# Autodesk Inventor assembly: coil winder V2
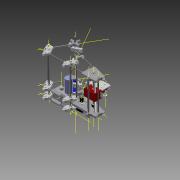
[picture p0: Inventor's stored thumbnail of the model, 180x180]
Saved by Autodesk Inventor 2013 (Build 170138000, 138)
## iProperties
Created: 2013-01-01
Part Number: coil winder V2
Document SubType Name: Assembly
Designer: Nico
Mass: 1980.92 g
Surface Area: 5858.81 cm^2
Volume: 1384.16 cm^3
Density: 1.43114 g/cm^3
Author: Nico
## Documents named in this file (37)
- D:\Documents\Inventor\Coil winder\IAM files\coil winder V2.iam
- D:\Documents\Inventor\Coil winder\IAM files\Winder Assembly 1.iam
- D:\Documents\Inventor\Coil winder\Drive thread.ipt
- D:\Documents\Inventor\Coil winder\IPT files\Washer M8.ipt
- D:\Documents\Inventor\Coil winder\IPT files\Half Nut M8.ipt
- D:\Documents\Inventor\Coil winder\IPT files\Pulley HTD 3-40-7.8.ipt
- D:\Documents\Inventor\Coil winder\IPT files\DC Motor stand V2.ipt
- D:\Documents\Inventor\Coil winder\IAM files\Nut+Washer M8.iam
- D:\Documents\Inventor\Coil winder\IAM files\Motor assembly V2.iam
- D:\Documents\Inventor\Coil winder\IPT files\carre Washer M8.ipt
- D:\Documents\Inventor\Coil winder\IPT files\bolt M4 x 10 nickel plated.ipt
- D:\Documents\Inventor\Coil winder\IPT files\connect stepper.ipt
- D:\Documents\Inventor\Coil winder\coil winder V2\Design Accelerator\Compress Spring1.iam
- D:\Documents\Inventor\Coil winder\IPT files\Sensor stand.ipt
- D:\Documents\Inventor\Coil winder\IPT files\optical sensor pcb.ipt
- D:\Documents\Inventor\Coil winder\IPT files\Vertex Bottom tensioner left.ipt
- D:\Documents\Inventor\Coil winder\IPT files\slide rod.ipt
- D:\Documents\Inventor\Coil winder\IAM files\Wire tension assembly.iam
- D:\Documents\Inventor\Coil winder\IPT files\608ZZ bearing.ipt
- D:\Documents\Inventor\Coil winder\IPT files\Nema 17 stepper motor.ipt
- D:\Documents\Inventor\Coil winder\Drive thread\Thread rod M8 x 100 mm.ipt
- D:\Documents\Inventor\Coil winder\Drive thread\Thread rod M8 x 300 mm.ipt
- D:\Documents\Inventor\Coil winder\Drive thread\Thread rod M8 x 190 mm.ipt
- D:\Documents\Inventor\Coil winder\Drive thread\Thread rod M8 x 250 mm.ipt
- D:\Documents\Inventor\Coil winder\IPT files\Vertex Bottom tensioner right.ipt
- D:\Documents\Inventor\Coil winder\Drive thread\Thread rod M8 x 380 mm.ipt
- D:\Documents\Inventor\Coil winder\Drive thread\Thread rod M8 x 230 mm.ipt
- D:\Documents\Inventor\Coil winder\IPT files\Stepper Pulley HTD 3 x 6 x 20.ipt
- D:\Documents\Inventor\Coil winder\IPT files\bolt M3 x 12 nickel plated.ipt
- D:\Documents\Inventor\Coil winder\IPT files\Washer M3 nickel plated.ipt
- D:\Documents\Inventor\Coil winder\IPT files\Tensioner Pulley HTD 3 x 6 x 20.ipt
- D:\Documents\Inventor\Coil winder\IPT files\Coil Coupling_1.ipt
- D:\Documents\Inventor\Coil winder\IPT files\Coil Coupling_2.ipt
- D:\Documents\Inventor\Coil winder\Drive thread\8mm thread 150 mm long.ipt
- D:\Documents\Inventor\Coil winder\IPT files\Drive thread.ipt
- D:\Documents\Inventor\Coil winder\IPT files\coil tightner.ipt
- Stepper Pulley HTD 3 x 6 x 20.ipt
## Components (151 placed, 32 different names)
1. Winder Assembly 1:1 [sub-assembly] — Mate:1, Mate:2, Mate:17, Mate:18, Mate:46, Mate:47, Mate:60, Mate:61, Mate:65, Mate:88, Mate:89, Mate:96, Mate:98, Mate:145, Flush:8, Mate:151, Mate:152, Mate:179, Mate:181, Mate:212, Mate:216, Mate:227, Mate:228
2. Winder Assembly 1:2 [sub-assembly] — Mate:1, Mate:2, Mate:4, Mate:19, Mate:20, Mate:30, Mate:42, Mate:43, Mate:62, Mate:63, Mate:64, Mate:72, Mate:73, Mate:80, Mate:81, Mate:180, Mate:210, Mate:215, Mate:225, Mate:226
3. Thread rod M8 x 100 mm:1 — Mate:4, Mate:13, Mate:14, Mate:15, Mate:16, Flush:1, Mate:21, Mate:27, Mate:100, Mate:114, Mate:137
4. Washer M8:1 — Mate:5, Mate:9, Mate:17
5. Washer M8:2 — Mate:6, Mate:12, Mate:20
6. Washer M8:3 — Mate:7, Mate:10, Mate:19
7. Washer M8:4 — Mate:8, Mate:11, Mate:18
8. Half Nut M8:1 — Mate:5, Mate:9, Mate:13
9. Half Nut M8:2 — Mate:6, Mate:12, Mate:14, Flush:1
10. Half Nut M8:3 — Mate:7, Mate:10, Mate:15, Mate:29
11. Half Nut M8:4 — Mate:8, Mate:11, Mate:16, Mate:140
12. Pulley HTD 3-40-7.8:1 — Mate:21, Mate:28, Mate:115
13. Washer M8:5 — Mate:23, Mate:25, Mate:115
14. Washer M8:6 — Mate:28, Mate:29, Mate:114
15. Half Nut M8:5 — Mate:23, Mate:25, Mate:27
16. Thread rod M8 x 300 mm:3 — Mate:30, Mate:52, Mate:53, Mate:58, Mate:59, Flush:3, Mate:99, Mate:126, Mate:127
17. Washer M8:7 — Mate:33, Mate:38, Mate:43
18. Washer M8:8 — Mate:35, Mate:37, Mate:47
19. Washer M8:9 — Mate:48, Mate:49, Mate:60
20. Washer M8:10 — Mate:54, Mate:55, Mate:61
21. Washer M8:11 — Mate:32, Mate:39, Mate:42
22. Washer M8:12 — Mate:34, Mate:36, Mate:46
23. Washer M8:13 — Mate:50, Mate:51, Mate:63
24. Washer M8:14 — Mate:56, Mate:57, Mate:62
25. Half Nut M8:6 — Mate:32, Mate:39
26. Half Nut M8:7 — Mate:33, Mate:38
27. Half Nut M8:8 — Mate:34, Mate:36
28. Half Nut M8:9 — Mate:35, Mate:37
29. Half Nut M8:10 — Mate:50, Mate:51, Mate:52, Flush:3
30. Half Nut M8:11 — Mate:48, Mate:49, Mate:53
31. Half Nut M8:12 — Mate:54, Mate:55, Mate:59
32. Half Nut M8:13 — Mate:56, Mate:57, Mate:58
33. Thread rod M8 x 190 mm:4 — Mate:64, Mate:70, Mate:71, Flush:4, Mate:78, Mate:79, Mate:102
34. Thread rod M8 x 380 mm:5 — Mate:65, Mate:86, Mate:87, Mate:95, Mate:97, Mate:101, Mate:282, Flush:33, Mate:429, Flush:34
35. Half Nut M8:14 — Mate:75, Mate:76, Mate:78
36. Half Nut M8:15 — Mate:74, Mate:77, Mate:79
37. Half Nut M8:16 — Mate:66, Mate:69, Mate:70
38. Half Nut M8:17 — Mate:67, Mate:68, Mate:71, Flush:4
39. Washer M8:15 — Mate:75, Mate:76, Mate:80
40. Washer M8:16 — Mate:74, Mate:77, Mate:81
41. Washer M8:17 — Mate:66, Mate:69, Mate:72
42. Washer M8:18 — Mate:67, Mate:68, Mate:73
43. Washer M8:19 — Mate:91, Mate:92, Mate:98
44. Washer M8:20 — Mate:90, Mate:93, Mate:96
45. Washer M8:21 — Mate:82, Mate:84, Mate:88
46. Washer M8:22 — Mate:83, Mate:85, Mate:89
47. Half Nut M8:18 — Mate:91, Mate:92, Mate:97, Flush:33
48. Half Nut M8:19 — Mate:90, Mate:93, Mate:95
49. Half Nut M8:20 — Mate:82, Mate:84, Mate:87
50. Half Nut M8:21 — Mate:83, Mate:85, Mate:86
51. Winder Assembly 1:3 [sub-assembly] — Mate:99, Mate:100, Mate:117, Mate:122, Mate:123, Mate:124, Mate:125, Mate:130, Mate:131, Mate:132, Mate:133, Mate:165, Mate:169, Mate:182, Mate:184, Mate:206, Mate:208, Mate:219, Mate:220, Mate:392, Mate:394, Mate:396
52. DC Motor stand V2:1 — Mate:101, Mate:102, Mate:103, Mate:105, Mate:106, Mate:107, Mate:108, Mate:109, Mate:110, Mate:113, Mate:422, Mate:423
53. Nut+Washer M8:1 [sub-assembly] — Mate:105, Mate:107
54. Nut+Washer M8:2 [sub-assembly] — Mate:106, Mate:109
55. Nut+Washer M8:3 [sub-assembly] — Mate:104, Mate:110
56. Nut+Washer M8:4 [sub-assembly] — Mate:103, Mate:104, Mate:108
57. Motor assembly V2:1 [sub-assembly] — Mate:113, Mate:422, Mate:423, Mate:424, Mate:425, Mate:426, Mate:427
58. Thread rod M8 x 380 mm:6 — Mate:117, Mate:118, Mate:119, Mate:120, Mate:121, Flush:6, Mate:231, Mate:232, Mate:402
59. Nut+Washer M8:5 [sub-assembly] — Mate:118, Mate:125
60. Nut+Washer M8:6 [sub-assembly] — Mate:120, Mate:123, Flush:6
61. Nut+Washer M8:7 [sub-assembly] — Mate:121, Mate:122
62. Nut+Washer M8:8 [sub-assembly] — Mate:119, Mate:124
63. Nut+Washer M8:9 [sub-assembly] — Mate:126, Mate:133
64. Nut+Washer M8:10 [sub-assembly] — Mate:127, Mate:132
65. Nut+Washer M8:11 [sub-assembly] — Mate:131, Mate:183, Flush:19
66. Nut+Washer M8:12 [sub-assembly] — Mate:130, Mate:287
67. Coil Coupling_1:1 — Mate:470
68. Half Nut M8:22 — Mate:137, Mate:138
69. Washer M8:23 — Mate:138, Mate:140
70. Bolt M4 x 10 nickel plated:1 — Mate:424, Mate:426
71. Bolt M4 x 10 nickel plated:2 — Mate:425, Mate:427
72. connect stepper:1 — Mate:145, Flush:8, Mate:146, Mate:148, Mate:149, Mate:150, Mate:153, Mate:154, Flush:32
73. Thread rod M8 x 230 mm:7 — Mate:146, Mate:147, Flush:9, Mate:274, Mate:281
74. Nut+Washer M8:13 [sub-assembly] — Mate:147, Mate:150
75. Nut+Washer M8:14 [sub-assembly] — Mate:148, Mate:149, Flush:9
76. Nut+Washer M8:15 [sub-assembly] — Mate:152, Mate:153
77. Nut+Washer M8:16 [sub-assembly] — Mate:151, Mate:154
78. connect stepper:2 — Mate:392, Mate:395, Mate:397, Mate:398, Mate:399, Mate:400, Flush:32
79. Thread rod M8 x 230 mm:8 — Mate:157, Mate:158, Flush:12, Mate:233, Mate:398, Mate:401, Mate:404
80. Nut+Washer M8:17 [sub-assembly] — Mate:157, Mate:400
81. Nut+Washer M8:18 [sub-assembly] — Mate:158, Flush:12, Mate:399
82. Nut+Washer M8:19 [sub-assembly] — Mate:394, Mate:397
83. Nut+Washer M8:20 [sub-assembly] — Mate:395, Mate:396
84. 8mm thread 150 mm long:16 — Mate:165, Mate:166, Mate:172, Mate:173, Mate:175, Mate:468, Mate:469, Mate:471
85. Nut+Washer M8:21 [sub-assembly] — Mate:166, Mate:169
86. Coil Coupling_1:2
87. Half Nut M8:23 — Mate:172
88. Washer M8:24 — Mate:173, Flush:14
89. Compress Spring:1 [sub-assembly] — Mate:175, Flush:14
90. Sensor stand:1 — Mate:179, Mate:180
91. optical sensor pcb:1
92. Thread rod M8 x 300 mm:10 — Mate:181, Mate:205, Flush:16, Mate:207, Mate:209, Mate:211, Mate:213, Mate:214, Flush:17
93. Thread rod M8 x 300 mm:11 — Mate:182, Mate:217, Mate:218, Flush:18, Mate:221, Mate:222, Mate:223, Mate:224, Flush:20
94. Thread rod M8 x 300 mm:12 — Mate:183, Mate:184, Flush:19, Mate:287
95. Vertex Bottom tensioner left:1 — Mate:401, Mate:402, Mate:403, Mate:405, Mate:406, Mate:407, Mate:408, Mate:409, Mate:410, Mate:411, Mate:412, Mate:413, Mate:414, Mate:415, Mate:416, Mate:417, Mate:420, Mate:421
96. Thread rod M8 x 250 mm:13 — Mate:238, Mate:241, Mate:244, Flush:23, Mate:264, Mate:269, Mate:412
97. slide rod:1 — Mate:410, Mate:415, Mate:419
98. slide rod:2 — Mate:411, Mate:416, Mate:418
99. 608ZZ bearing:1 — Mate:204, Mate:249, Mate:250, Mate:414
100. 608ZZ bearing:2 — Mate:279, Mate:280, Mate:430, Mate:431
101. Thread rod M8 x 250 mm:14 — Mate:204, Mate:247, Mate:248, Flush:24, Mate:272, Mate:275, Mate:409, Mate:430, Mate:434, Mate:444, Mate:445
102. Nut+Washer M8:23 [sub-assembly] — Mate:205, Mate:206, Flush:16
103. Nut+Washer M8:24 [sub-assembly] — Mate:218, Mate:220
104. Nut+Washer M8:25 [sub-assembly] — Mate:207, Mate:208
105. Nut+Washer M8:26 [sub-assembly] — Mate:217, Mate:219, Flush:18
106. Nut+Washer M8:27 [sub-assembly] — Mate:209, Mate:210, Flush:17
107. Nut+Washer M8:28 [sub-assembly] — Mate:211, Mate:212
108. Nut+Washer M8:29 [sub-assembly] — Mate:214, Mate:215
109. Nut+Washer M8:30 [sub-assembly] — Mate:213, Mate:216
110. Nut+Washer M8:31 [sub-assembly] — Mate:221, Mate:227
111. Nut+Washer M8:32 [sub-assembly] — Mate:222, Mate:228
112. Nut+Washer M8:33 [sub-assembly] — Mate:223, Mate:226, Flush:20
113. Nut+Washer M8:34 [sub-assembly] — Mate:224, Mate:225
114. Nut+Washer M8:35 [sub-assembly] — Mate:404, Mate:405
115. Nut+Washer M8:36 [sub-assembly] — Mate:231, Mate:421
116. Nut+Washer M8:37 [sub-assembly] — Mate:232, Mate:403
117. Nut+Washer M8:38 [sub-assembly] — Mate:233, Mate:406
118. Thread rod M8 x 250 mm:15 — Mate:239, Mate:242, Flush:22, Mate:266, Mate:268, Mate:407
119. Nut+Washer M8:39 [sub-assembly] — Mate:238, Flush:23, Mate:413
120. Nut+Washer M8:40 [sub-assembly] — Mate:239, Flush:22, Mate:417
121. Nut+Washer M8:41 [sub-assembly] — Mate:241, Mate:244, Mate:420
122. Nut+Washer M8:42 [sub-assembly] — Mate:242, Mate:408
123. Nut+Washer M8:43 [sub-assembly] — Mate:247, Mate:250, Flush:24
124. Nut+Washer M8:44 [sub-assembly] — Mate:248, Mate:249
125. Nut+Washer M8:45 [sub-assembly] — Mate:266, Mate:435
126. Nut+Washer M8:46 [sub-assembly] — Mate:264, Mate:438, Mate:439
127. Nut+Washer M8:47 [sub-assembly] — Mate:269, Mate:437
128. Nut+Washer M8:48 [sub-assembly] — Mate:268, Mate:436
129. Nut+Washer M8:49 [sub-assembly] — Mate:274
130. Nut+Washer M8:51 [sub-assembly] — Mate:275, Mate:280
131. Nut+Washer M8:52 [sub-assembly] — Mate:272, Mate:279
132. Nut+Washer M8:53 [sub-assembly] — Mate:281, Mate:433
133. Nut+Washer M8:54 [sub-assembly] — Mate:282, Mate:432, Flush:34
134. Wire tension assembly:1 [sub-assembly] — Mate:418, Mate:419
135. Nema 17 stepper motor:1 — Mate:434, Flush:35, Mate:449, Mate:462, Mate:463, Mate:464, Mate:465
136. Vertex Bottom tensioner right:1 — Mate:429, Mate:431, Mate:432, Mate:433, Mate:435, Mate:436, Mate:437, Mate:438, Mate:439, Flush:35, Mate:458, Mate:459, Mate:460, Mate:461
137. Stepper Pulley HTD 3 x 6 x 20:1 — Mate:449
138. Tensioner Pulley HTD 3 x 6 x 20:1
139. Nut+Washer M8:55 [sub-assembly] — Mate:445
140. Nut+Washer M8:56 [sub-assembly] — Mate:444
141. bolt M3 x 12 nickel plated:1 — Mate:453, Mate:456, Mate:463
142. bolt M3 x 12 nickel plated:2 — Mate:450, Mate:455, Mate:462
143. bolt M3 x 12 nickel plated:3 — Mate:451, Mate:454, Mate:465
144. bolt M3 x 12 nickel plated:4 — Mate:452, Mate:457, Mate:464
145. Washer M3 Nickel plated:1 — Mate:453, Mate:456, Mate:459
146. Washer M3 Nickel plated:2 — Mate:452, Mate:457, Mate:460
147. Washer M3 Nickel plated:3 — Mate:451, Mate:454, Mate:461
148. Washer M3 Nickel plated:4 — Mate:450, Mate:455, Mate:458
149. Coil Coupling_2:1 — Mate:468
150. Coil Coupling_2:2 — Mate:469, Mate:470
151. coil tightner:1 — Mate:471
## Relationships (286: Mate 266, Flush 20)
- Mate:1: Winder Assembly 1:1 ↔ Winder Assembly 1:2
- Mate:2: Winder Assembly 1:1 ↔ Winder Assembly 1:2
- Mate:4: Winder Assembly 1:2 ↔ Thread rod M8 x 100 mm:1
- Mate:5: Washer M8:1 ↔ Half Nut M8:1
- Mate:6: Washer M8:2 ↔ Half Nut M8:2
- Mate:7: Washer M8:3 ↔ Half Nut M8:3
- Mate:8: Washer M8:4 ↔ Half Nut M8:4
- Mate:9: Washer M8:1 ↔ Half Nut M8:1
- Mate:10: Washer M8:3 ↔ Half Nut M8:3
- Mate:11: Washer M8:4 ↔ Half Nut M8:4
- Mate:12: Washer M8:2 ↔ Half Nut M8:2
- Mate:13: Thread rod M8 x 100 mm:1 ↔ Half Nut M8:1
- Mate:14: Thread rod M8 x 100 mm:1 ↔ Half Nut M8:2
- Mate:15: Thread rod M8 x 100 mm:1 ↔ Half Nut M8:3
- Mate:16: Thread rod M8 x 100 mm:1 ↔ Half Nut M8:4
- Mate:17: Winder Assembly 1:1 ↔ Washer M8:1
- Mate:18: Winder Assembly 1:1 ↔ Washer M8:4
- Mate:19: Winder Assembly 1:2 ↔ Washer M8:3
- Mate:20: Winder Assembly 1:2 ↔ Washer M8:2
- Flush:1 (-2 mm): Thread rod M8 x 100 mm:1 ↔ Half Nut M8:2
- Mate:21: Thread rod M8 x 100 mm:1 ↔ Pulley HTD 3-40-7.8:1
- Mate:23: Washer M8:5 ↔ Half Nut M8:5
- Mate:25: Washer M8:5 ↔ Half Nut M8:5
- Mate:27: Thread rod M8 x 100 mm:1 ↔ Half Nut M8:5
- Mate:28: Pulley HTD 3-40-7.8:1 ↔ Washer M8:6
- Mate:29: Half Nut M8:3 ↔ Washer M8:6
- Mate:30: Winder Assembly 1:2 ↔ Thread rod M8 x 300 mm:3
- Mate:32: Washer M8:11 ↔ Half Nut M8:6
- Mate:33: Washer M8:7 ↔ Half Nut M8:7
- Mate:34: Washer M8:12 ↔ Half Nut M8:8
- Mate:35: Washer M8:8 ↔ Half Nut M8:9
- Mate:36: Washer M8:12 ↔ Half Nut M8:8
- Mate:37: Washer M8:8 ↔ Half Nut M8:9
- Mate:38: Washer M8:7 ↔ Half Nut M8:7
- Mate:39: Washer M8:11 ↔ Half Nut M8:6
- Mate:42: Winder Assembly 1:2 ↔ Washer M8:11
- Mate:43: Winder Assembly 1:2 ↔ Washer M8:7
- Mate:46: Winder Assembly 1:1 ↔ Washer M8:12
- Mate:47: Winder Assembly 1:1 ↔ Washer M8:8
- Mate:48: Washer M8:9 ↔ Half Nut M8:11
- Mate:49: Washer M8:9 ↔ Half Nut M8:11
- Mate:50: Washer M8:13 ↔ Half Nut M8:10
- Mate:51: Washer M8:13 ↔ Half Nut M8:10
- Mate:52: Thread rod M8 x 300 mm:3 ↔ Half Nut M8:10
- Mate:53: Thread rod M8 x 300 mm:3 ↔ Half Nut M8:11
- Mate:54: Washer M8:10 ↔ Half Nut M8:12
- Mate:55: Washer M8:10 ↔ Half Nut M8:12
- Mate:56: Washer M8:14 ↔ Half Nut M8:13
- Mate:57: Washer M8:14 ↔ Half Nut M8:13
- Mate:58: Thread rod M8 x 300 mm:3 ↔ Half Nut M8:13
- Mate:59: Thread rod M8 x 300 mm:3 ↔ Half Nut M8:12
- Mate:60: Winder Assembly 1:1 ↔ Washer M8:9
- Mate:61: Winder Assembly 1:1 ↔ Washer M8:10
- Mate:62: Winder Assembly 1:2 ↔ Washer M8:14
- Mate:63: Winder Assembly 1:2 ↔ Washer M8:13
- Flush:3 (-2 mm): Thread rod M8 x 300 mm:3 ↔ Half Nut M8:10
- Mate:64: Winder Assembly 1:2 ↔ Thread rod M8 x 190 mm:4
- Mate:65: Winder Assembly 1:1 ↔ Thread rod M8 x 380 mm:5
- Mate:66: Half Nut M8:16 ↔ Washer M8:17
- Mate:67: Half Nut M8:17 ↔ Washer M8:18
- Mate:68: Half Nut M8:17 ↔ Washer M8:18
- Mate:69: Half Nut M8:16 ↔ Washer M8:17
- Mate:70: Thread rod M8 x 190 mm:4 ↔ Half Nut M8:16
- Mate:71: Thread rod M8 x 190 mm:4 ↔ Half Nut M8:17
- Mate:72: Winder Assembly 1:2 ↔ Washer M8:17
- Mate:73: Winder Assembly 1:2 ↔ Washer M8:18
- Flush:4 (-2 mm): Thread rod M8 x 190 mm:4 ↔ Half Nut M8:17
- Mate:74: Half Nut M8:15 ↔ Washer M8:16
- Mate:75: Half Nut M8:14 ↔ Washer M8:15
- Mate:76: Half Nut M8:14 ↔ Washer M8:15
- Mate:77: Half Nut M8:15 ↔ Washer M8:16
- Mate:78: Thread rod M8 x 190 mm:4 ↔ Half Nut M8:14
- Mate:79: Thread rod M8 x 190 mm:4 ↔ Half Nut M8:15
- Mate:80: Winder Assembly 1:2 ↔ Washer M8:15
- Mate:81: Winder Assembly 1:2 ↔ Washer M8:16
- Mate:82: Washer M8:21 ↔ Half Nut M8:20
- Mate:83: Washer M8:22 ↔ Half Nut M8:21
- Mate:84: Washer M8:21 ↔ Half Nut M8:20
- Mate:85: Washer M8:22 ↔ Half Nut M8:21
- Mate:86: Thread rod M8 x 380 mm:5 ↔ Half Nut M8:21
- Mate:87: Thread rod M8 x 380 mm:5 ↔ Half Nut M8:20
- Mate:88: Winder Assembly 1:1 ↔ Washer M8:21
- Mate:89: Winder Assembly 1:1 ↔ Washer M8:22
- Mate:90: Washer M8:20 ↔ Half Nut M8:19
- Mate:91: Washer M8:19 ↔ Half Nut M8:18
- Mate:92: Washer M8:19 ↔ Half Nut M8:18
- Mate:93: Washer M8:20 ↔ Half Nut M8:19
- Mate:95: Thread rod M8 x 380 mm:5 ↔ Half Nut M8:19
- Mate:96: Winder Assembly 1:1 ↔ Washer M8:20
- Mate:97: Thread rod M8 x 380 mm:5 ↔ Half Nut M8:18
- Mate:98: Winder Assembly 1:1 ↔ Washer M8:19
- Mate:99: Thread rod M8 x 300 mm:3 ↔ Winder Assembly 1:3
- Mate:100: Thread rod M8 x 100 mm:1 ↔ Winder Assembly 1:3
- Mate:101: Thread rod M8 x 380 mm:5 ↔ DC Motor stand V2:1
- Mate:102: Thread rod M8 x 190 mm:4 ↔ DC Motor stand V2:1
- Mate:103: DC Motor stand V2:1 ↔ Nut+Washer M8:4
- Mate:104: Nut+Washer M8:3 ↔ Nut+Washer M8:4
- Mate:105: DC Motor stand V2:1 ↔ Nut+Washer M8:1
- Mate:106: DC Motor stand V2:1 ↔ Nut+Washer M8:2
- Mate:107: DC Motor stand V2:1 ↔ Nut+Washer M8:1
- Mate:108: DC Motor stand V2:1 ↔ Nut+Washer M8:4
- Mate:109: DC Motor stand V2:1 ↔ Nut+Washer M8:2
- Mate:110: DC Motor stand V2:1 ↔ Nut+Washer M8:3
- Mate:113: DC Motor stand V2:1 ↔ Motor assembly V2:1
- Mate:114: Thread rod M8 x 100 mm:1 ↔ Washer M8:6
- Mate:115: Pulley HTD 3-40-7.8:1 ↔ Washer M8:5
- Mate:117: Winder Assembly 1:3 ↔ Thread rod M8 x 380 mm:6
- Mate:118: Thread rod M8 x 380 mm:6 ↔ Nut+Washer M8:5
- Mate:119: Thread rod M8 x 380 mm:6 ↔ Nut+Washer M8:8
- Mate:120: Thread rod M8 x 380 mm:6 ↔ Nut+Washer M8:6
- Mate:121: Thread rod M8 x 380 mm:6 ↔ Nut+Washer M8:7
- Mate:122: Winder Assembly 1:3 ↔ Nut+Washer M8:7
- Mate:123: Winder Assembly 1:3 ↔ Nut+Washer M8:6
- Mate:124: Winder Assembly 1:3 ↔ Nut+Washer M8:8
- Mate:125: Winder Assembly 1:3 ↔ Nut+Washer M8:5
- Flush:6 (-2 mm): Thread rod M8 x 380 mm:6 ↔ Nut+Washer M8:6
- Mate:126: Thread rod M8 x 300 mm:3 ↔ Nut+Washer M8:9
- Mate:127: Thread rod M8 x 300 mm:3 ↔ Nut+Washer M8:10
- Mate:130: Winder Assembly 1:3 ↔ Nut+Washer M8:12
- Mate:131: Winder Assembly 1:3 ↔ Nut+Washer M8:11
- Mate:132: Winder Assembly 1:3 ↔ Nut+Washer M8:10
- Mate:133: Winder Assembly 1:3 ↔ Nut+Washer M8:9
- Mate:137: Thread rod M8 x 100 mm:1 ↔ Half Nut M8:22
- Mate:138: Half Nut M8:22 ↔ Washer M8:23
- Mate:140: Half Nut M8:4 ↔ Washer M8:23
- Mate:145: Winder Assembly 1:1 ↔ connect stepper:1
- Flush:8 (-0.5 mm): Winder Assembly 1:1 ↔ connect stepper:1
- Mate:146: connect stepper:1 ↔ Thread rod M8 x 230 mm:7
- Mate:147: Thread rod M8 x 230 mm:7 ↔ Nut+Washer M8:13
- Mate:148: connect stepper:1 ↔ Nut+Washer M8:14
- Mate:149: connect stepper:1 ↔ Nut+Washer M8:14
- Mate:150: connect stepper:1 ↔ Nut+Washer M8:13
- Flush:9 (-2 mm): Thread rod M8 x 230 mm:7 ↔ Nut+Washer M8:14
- Mate:151: Winder Assembly 1:1 ↔ Nut+Washer M8:16
- Mate:152: Winder Assembly 1:1 ↔ Nut+Washer M8:15
- Mate:153: connect stepper:1 ↔ Nut+Washer M8:15
- Mate:154: connect stepper:1 ↔ Nut+Washer M8:16
- Mate:157: Thread rod M8 x 230 mm:8 ↔ Nut+Washer M8:17
- Mate:158: Thread rod M8 x 230 mm:8 ↔ Nut+Washer M8:18
- Flush:12 (-2 mm): Thread rod M8 x 230 mm:8 ↔ Nut+Washer M8:18
- Mate:165: Winder Assembly 1:3 ↔ 8mm thread 150 mm long:16
- Mate:166: 8mm thread 150 mm long:16 ↔ Nut+Washer M8:21
- Mate:169: Winder Assembly 1:3 ↔ Nut+Washer M8:21
- Mate:172: 8mm thread 150 mm long:16 ↔ Half Nut M8:23
- Mate:173: 8mm thread 150 mm long:16 ↔ Washer M8:24
- Mate:175: 8mm thread 150 mm long:16 ↔ Compress Spring:1
- Flush:14: Washer M8:24 ↔ Compress Spring:1
- Mate:179: Winder Assembly 1:1 ↔ Sensor stand:1
- Mate:180: Winder Assembly 1:2 ↔ Sensor stand:1
- Mate:181: Winder Assembly 1:1 ↔ Thread rod M8 x 300 mm:10
- Mate:182: Winder Assembly 1:3 ↔ Thread rod M8 x 300 mm:11
- Mate:183: Nut+Washer M8:11 ↔ Thread rod M8 x 300 mm:12
- Mate:184: Winder Assembly 1:3 ↔ Thread rod M8 x 300 mm:12
- Mate:204: 608ZZ bearing:1 ↔ Thread rod M8 x 250 mm:14
- Mate:205: Thread rod M8 x 300 mm:10 ↔ Nut+Washer M8:23
- Mate:206: Winder Assembly 1:3 ↔ Nut+Washer M8:23
- Flush:16 (-2 mm): Thread rod M8 x 300 mm:10 ↔ Nut+Washer M8:23
- Mate:207: Thread rod M8 x 300 mm:10 ↔ Nut+Washer M8:25
- Mate:208: Winder Assembly 1:3 ↔ Nut+Washer M8:25
- Mate:209: Thread rod M8 x 300 mm:10 ↔ Nut+Washer M8:27
- Mate:210: Winder Assembly 1:2 ↔ Nut+Washer M8:27
- Mate:211: Thread rod M8 x 300 mm:10 ↔ Nut+Washer M8:28
- Mate:212: Winder Assembly 1:1 ↔ Nut+Washer M8:28
- Mate:213: Thread rod M8 x 300 mm:10 ↔ Nut+Washer M8:30
- Mate:214: Thread rod M8 x 300 mm:10 ↔ Nut+Washer M8:29
- Mate:215: Winder Assembly 1:2 ↔ Nut+Washer M8:29
- Mate:216: Winder Assembly 1:1 ↔ Nut+Washer M8:30
- Flush:17 (-2 mm): Thread rod M8 x 300 mm:10 ↔ Nut+Washer M8:27
- Mate:217: Thread rod M8 x 300 mm:11 ↔ Nut+Washer M8:26
- Mate:218: Thread rod M8 x 300 mm:11 ↔ Nut+Washer M8:24
- Mate:219: Winder Assembly 1:3 ↔ Nut+Washer M8:26
- Mate:220: Winder Assembly 1:3 ↔ Nut+Washer M8:24
- Flush:18 (-2 mm): Thread rod M8 x 300 mm:11 ↔ Nut+Washer M8:26
- Flush:19 (-2 mm): Nut+Washer M8:11 ↔ Thread rod M8 x 300 mm:12
- Mate:221: Thread rod M8 x 300 mm:11 ↔ Nut+Washer M8:31
- Mate:222: Thread rod M8 x 300 mm:11 ↔ Nut+Washer M8:32
- Mate:223: Thread rod M8 x 300 mm:11 ↔ Nut+Washer M8:33
- Mate:224: Thread rod M8 x 300 mm:11 ↔ Nut+Washer M8:34
- Mate:225: Winder Assembly 1:2 ↔ Nut+Washer M8:34
- Mate:226: Winder Assembly 1:2 ↔ Nut+Washer M8:33
- Flush:20 (-2 mm): Thread rod M8 x 300 mm:11 ↔ Nut+Washer M8:33
- Mate:227: Winder Assembly 1:1 ↔ Nut+Washer M8:31
- Mate:228: Winder Assembly 1:1 ↔ Nut+Washer M8:32
- Mate:231: Thread rod M8 x 380 mm:6 ↔ Nut+Washer M8:36
- Mate:232: Thread rod M8 x 380 mm:6 ↔ Nut+Washer M8:37
- Mate:233: Thread rod M8 x 230 mm:8 ↔ Nut+Washer M8:38
- Mate:238: Thread rod M8 x 250 mm:13 ↔ Nut+Washer M8:39
- Mate:239: Thread rod M8 x 250 mm:15 ↔ Nut+Washer M8:40
- Mate:241: Thread rod M8 x 250 mm:13 ↔ Nut+Washer M8:41
- Mate:242: Thread rod M8 x 250 mm:15 ↔ Nut+Washer M8:42
- Mate:244: Thread rod M8 x 250 mm:13 ↔ Nut+Washer M8:41
- Flush:22 (-2 mm): Thread rod M8 x 250 mm:15 ↔ Nut+Washer M8:40
- Flush:23 (-2 mm): Thread rod M8 x 250 mm:13 ↔ Nut+Washer M8:39
- Mate:247: Thread rod M8 x 250 mm:14 ↔ Nut+Washer M8:43
- Mate:248: Thread rod M8 x 250 mm:14 ↔ Nut+Washer M8:44
- Mate:249: 608ZZ bearing:1 ↔ Nut+Washer M8:44
- Mate:250: 608ZZ bearing:1 ↔ Nut+Washer M8:43
- Flush:24 (-5 mm): Thread rod M8 x 250 mm:14 ↔ Nut+Washer M8:43
- Mate:264: Thread rod M8 x 250 mm:13 ↔ Nut+Washer M8:46
- Mate:266: Thread rod M8 x 250 mm:15 ↔ Nut+Washer M8:45
- Mate:268: Thread rod M8 x 250 mm:15 ↔ Nut+Washer M8:48
- Mate:269: Thread rod M8 x 250 mm:13 ↔ Nut+Washer M8:47
- Mate:272: Thread rod M8 x 250 mm:14 ↔ Nut+Washer M8:52
- Mate:274: Thread rod M8 x 230 mm:7 ↔ Nut+Washer M8:49
- Mate:275: Thread rod M8 x 250 mm:14 ↔ Nut+Washer M8:51
- Mate:279: 608ZZ bearing:2 ↔ Nut+Washer M8:52
- Mate:280: 608ZZ bearing:2 ↔ Nut+Washer M8:51
- Mate:281: Thread rod M8 x 230 mm:7 ↔ Nut+Washer M8:53
- Mate:282: Thread rod M8 x 380 mm:5 ↔ Nut+Washer M8:54
- Mate:287: Nut+Washer M8:12 ↔ Thread rod M8 x 300 mm:12
- Mate:392: Winder Assembly 1:3 ↔ connect stepper:2
- Mate:394: Winder Assembly 1:3 ↔ Nut+Washer M8:19
- Mate:395: connect stepper:2 ↔ Nut+Washer M8:20
- Mate:396: Winder Assembly 1:3 ↔ Nut+Washer M8:20
- Mate:397: connect stepper:2 ↔ Nut+Washer M8:19
- Mate:398: connect stepper:2 ↔ Thread rod M8 x 230 mm:8
- Mate:399: connect stepper:2 ↔ Nut+Washer M8:18
- Mate:400: connect stepper:2 ↔ Nut+Washer M8:17
- Mate:401: Thread rod M8 x 230 mm:8 ↔ Vertex Bottom tensioner left:1
- Mate:402: Thread rod M8 x 380 mm:6 ↔ Vertex Bottom tensioner left:1
- Mate:403: Vertex Bottom tensioner left:1 ↔ Nut+Washer M8:37
- Mate:404: Thread rod M8 x 230 mm:8 ↔ Nut+Washer M8:35
- Mate:405: Vertex Bottom tensioner left:1 ↔ Nut+Washer M8:35
- Mate:406: Vertex Bottom tensioner left:1 ↔ Nut+Washer M8:38
- Mate:407: Vertex Bottom tensioner left:1 ↔ Thread rod M8 x 250 mm:15
- Mate:408: Vertex Bottom tensioner left:1 ↔ Nut+Washer M8:42
- Mate:409: Vertex Bottom tensioner left:1 ↔ Thread rod M8 x 250 mm:14
- Mate:410: Vertex Bottom tensioner left:1 ↔ slide rod:1
- Mate:411: Vertex Bottom tensioner left:1 ↔ slide rod:2
- Mate:412: Vertex Bottom tensioner left:1 ↔ Thread rod M8 x 250 mm:13
- Mate:413: Vertex Bottom tensioner left:1 ↔ Nut+Washer M8:39
- Mate:414: Vertex Bottom tensioner left:1 ↔ 608ZZ bearing:1
- Mate:415: Vertex Bottom tensioner left:1 ↔ slide rod:1
- Mate:416: Vertex Bottom tensioner left:1 ↔ slide rod:2
- Mate:417: Vertex Bottom tensioner left:1 ↔ Nut+Washer M8:40
- Mate:418: slide rod:2 ↔ Wire tension assembly:1
- Mate:419: slide rod:1 ↔ Wire tension assembly:1
- Mate:420: Vertex Bottom tensioner left:1 ↔ Nut+Washer M8:41
- Mate:421: Vertex Bottom tensioner left:1 ↔ Nut+Washer M8:36
- Flush:32: connect stepper:1 ↔ connect stepper:2
- Flush:33 (-2 mm): Thread rod M8 x 380 mm:5 ↔ Half Nut M8:18
- Mate:422: DC Motor stand V2:1 ↔ Motor assembly V2:1
- Mate:423: DC Motor stand V2:1 ↔ Motor assembly V2:1
- Mate:424: Motor assembly V2:1 ↔ Bolt M4 x 10 nickel plated:1
- Mate:425: Motor assembly V2:1 ↔ Bolt M4 x 10 nickel plated:2
- Mate:426: Motor assembly V2:1 ↔ Bolt M4 x 10 nickel plated:1
- Mate:427: Motor assembly V2:1 ↔ Bolt M4 x 10 nickel plated:2
- Mate:429: Thread rod M8 x 380 mm:5 ↔ Vertex Bottom tensioner right:1
- Mate:430: 608ZZ bearing:2 ↔ Thread rod M8 x 250 mm:14
- Mate:431: 608ZZ bearing:2 ↔ Vertex Bottom tensioner right:1
- Mate:432: Nut+Washer M8:54 ↔ Vertex Bottom tensioner right:1
- Flush:34 (-2 mm): Thread rod M8 x 380 mm:5 ↔ Nut+Washer M8:54
- Mate:433: Nut+Washer M8:53 ↔ Vertex Bottom tensioner right:1
- Mate:434 (83.7544 mm): Thread rod M8 x 250 mm:14 ↔ Nema 17 stepper motor:1
- Mate:435: Nut+Washer M8:45 ↔ Vertex Bottom tensioner right:1
- Mate:436: Nut+Washer M8:48 ↔ Vertex Bottom tensioner right:1
- Mate:437: Nut+Washer M8:47 ↔ Vertex Bottom tensioner right:1
- Mate:438: Nut+Washer M8:46 ↔ Vertex Bottom tensioner right:1
- Mate:439: Nut+Washer M8:46 ↔ Vertex Bottom tensioner right:1
- Flush:35 (-21 mm): Nema 17 stepper motor:1 ↔ Vertex Bottom tensioner right:1
- Mate:444: Thread rod M8 x 250 mm:14 ↔ Nut+Washer M8:56
- Mate:445: Thread rod M8 x 250 mm:14 ↔ Nut+Washer M8:55
- [Mate]: Thread rod M8 x 250 mm:14 ↔ Tensioner Pulley HTD 3 x 6 x 20:1
- [Mate]: Tensioner Pulley HTD 3 x 6 x 20:1 ↔ Nut+Washer M8:56
- [Mate]: Tensioner Pulley HTD 3 x 6 x 20:1 ↔ Nut+Washer M8:55
- Mate:449: Nema 17 stepper motor:1 ↔ Stepper Pulley HTD 3 x 6 x 20:1
- Mate:450: bolt M3 x 12 nickel plated:2 ↔ Washer M3 Nickel plated:4
- Mate:451: bolt M3 x 12 nickel plated:3 ↔ Washer M3 Nickel plated:3
- Mate:452: bolt M3 x 12 nickel plated:4 ↔ Washer M3 Nickel plated:2
- Mate:453: bolt M3 x 12 nickel plated:1 ↔ Washer M3 Nickel plated:1
- Mate:454: bolt M3 x 12 nickel plated:3 ↔ Washer M3 Nickel plated:3
- Mate:455: bolt M3 x 12 nickel plated:2 ↔ Washer M3 Nickel plated:4
- Mate:456: bolt M3 x 12 nickel plated:1 ↔ Washer M3 Nickel plated:1
- Mate:457: bolt M3 x 12 nickel plated:4 ↔ Washer M3 Nickel plated:2
- Mate:458: Vertex Bottom tensioner right:1 ↔ Washer M3 Nickel plated:4
- Mate:459: Vertex Bottom tensioner right:1 ↔ Washer M3 Nickel plated:1
- Mate:460: Vertex Bottom tensioner right:1 ↔ Washer M3 Nickel plated:2
- Mate:461: Vertex Bottom tensioner right:1 ↔ Washer M3 Nickel plated:3
- Mate:462: Nema 17 stepper motor:1 ↔ bolt M3 x 12 nickel plated:2
- Mate:463: Nema 17 stepper motor:1 ↔ bolt M3 x 12 nickel plated:1
- Mate:464: Nema 17 stepper motor:1 ↔ bolt M3 x 12 nickel plated:4
- Mate:465: Nema 17 stepper motor:1 ↔ bolt M3 x 12 nickel plated:3
- Mate:468: 8mm thread 150 mm long:16 ↔ Coil Coupling_2:1
- Mate:469: 8mm thread 150 mm long:16 ↔ Coil Coupling_2:2
- Mate:470: Coil Coupling_1:1 ↔ Coil Coupling_2:2
- Mate:471: 8mm thread 150 mm long:16 ↔ coil tightner:1
